# Autodesk Inventor assembly: 2906-0006-0008 assembly
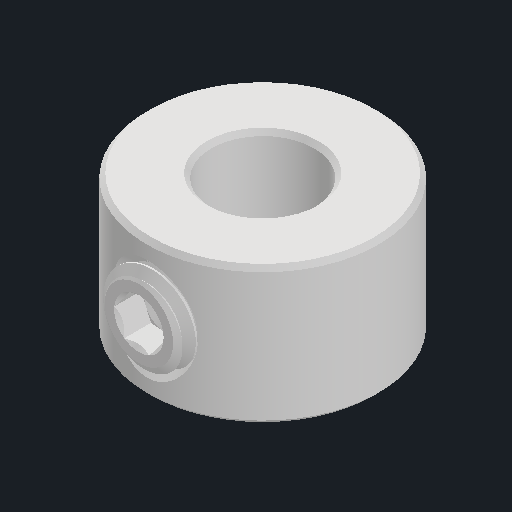
[picture p0: Inventor's stored thumbnail of the model, 512x512]
Saved by Autodesk Inventor 2023 (Build 270158000, 158)
## iProperties
Created: 2018-01-19
Part Number: 2906-0006-0008 assembly
Description: STEP AP203
Document SubType Name: Assembly
Designer: Arash
Sending System: SolidWorks 2016
Preprocessor: SwSTEP 2.0
Title: 2906-0006-0008 assembly.STEP
Revision Number: ANY
## Documents named in this file (3)
- c:\$workingfolder\Engineering Data\FTC_Parts_Library\goBilda\Motion\Collars\6mm D-Shaft Set Screw Collar.iam
- c:\$workingfolder\Engineering Data\FTC_Parts_Library\goBilda\Motion\Collars\Without Screw\2906-0006-0008.ipt
- c:\$workingfolder\Engineering Data\FTC_Parts_Library\goBilda\Hardware (goBilda specific)\Screws\Set Screws\M5 x 4 Set Screw.ipt
## Components (2 placed, 2 different names)
1. 2906-0006-0008_1 — Mate:1
2. 2806-0005-0004_91390A117_2 — Mate:1
## Relationships (1: Mate 1)
- Mate:1: 2906-0006-0008_1 ↔ 2806-0005-0004_91390A117_2
